# Autodesk Inventor assembly: BodyStructure
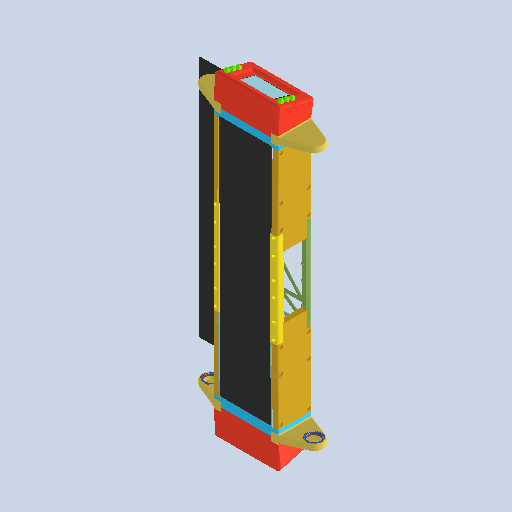
[picture p0: Inventor's stored thumbnail of the model, 512x512]
Saved by Autodesk Inventor 2023 (Build 270158000, 158)
## iProperties
Created: 2022-01-14
Part Number: BodyStructure
Document SubType Name: Assembly
Designer: Jochen
Author: Jochen
## Documents named in this file (13)
- D:\Projects\Lisbeth\CAD\BodyStructure.iam
- D:\Projects\Lisbeth\CAD\Body\BodyStructure Side.ipt
- D:\Projects\Lisbeth\CAD\Body\BodyStructure HipSupport.ipt
- D:\Projects\Lisbeth\CAD\Body\BodyStructure Centre Top.ipt
- D:\Projects\Lisbeth\CAD\Body\BodyStructure Plate.ipt
- D:\Projects\Lisbeth\CAD\Common\Bearing\bearing_27_20_4 s61704-2rsr.ipt
- D:\Projects\Lisbeth\CAD\Body\BodyCover.ipt
- D:\Projects\Lisbeth\CAD\Common\Accessories\Battery Pack.ipt
- D:\Projects\Lisbeth\CAD\Body\BodyStructure Centre Bottom.ipt
- D:\Projects\Lisbeth\CAD\Body\BodyStructure Head.ipt
- D:\Projects\Lisbeth\CAD\Body\BodyStructure Tail.ipt
- D:\Projects\Lisbeth\CAD\Common\Accessories\Adafruit 2.4 OLED display.ipt
- D:\Projects\Lisbeth\CAD\Common\Accessories\LED 5mm.ipt
## Components (28 placed, 10 different names)
1. BodyStructure Side:1 — Mate:89, Mate:100, Mate:102, Mate:142, Mate:149, Mate:150
2. BodyStructure Side:2 — Mate:109, Mate:110, Mate:111, Mate:138, Mate:139, Mate:140
3. BodyHipSupport:1 — Mate:38, Mate:39, Mate:153, Mate:154
4. BodyHipSupport:2 — Mate:44, Mate:45, Mate:151, Mate:152
5. Body Structure Centre Top:2 — Mate:46, Mate:95, Mate:115, Mate:116, Mate:138, Mate:140
6. BodyStructure Side:3 — Mate:46, Angle:2, Mate:139, Mate:141, Mate:143, Mate:144
7. BodyStructure Side:4 — Mate:101, Mate:115, Mate:142
8. BodyHipSupport:3 — Mate:42, Mate:43, Mate:145, Mate:146
9. BodyHipSupport:4 — Mate:40, Mate:41, Mate:147, Mate:148
10. bearing_27_20_4 s61704-2rsr:1 — Mate:38, Mate:39
11. bearing_27_20_4 s61704-2rsr:2 — Mate:44, Mate:45
12. bearing_27_20_4 s61704-2rsr:3 — Mate:40, Mate:41
13. bearing_27_20_4 s61704-2rsr:4 — Mate:42, Mate:43
14. BodyCover:1 — Mate:103, Mate:113
15. BodyCover:2 — Mate:95, Mate:116, Angle:1
16. Battery Pack 59x31x21:1 — Angle:1, Angle:2, Mate:159
17. Body Structure Centre:7 — Mate:89, Mate:109
18. Body Structure Centre Top:1 — Mate:100, Mate:101, Mate:102, Mate:103, Mate:113, Mate:141
19. Body Structure Centre:9 — Mate:110, Mate:111
20. BodyStructure Head:4 — Mate:143, Mate:144, Mate:145, Mate:146, Mate:147, Mate:148, Flush:1, Mate:156, Mate:157, Mate:158, Mate:159, Mate:160, Mate:161, Mate:162, Mate:163, Mate:164, Mate:165, Mate:166, Mate:167, Mate:168, Mate:169, Mate:170, Mate:171, Mate:172
21. BodyStructure Head:5 — Mate:149, Mate:150, Mate:151, Mate:152, Mate:153, Mate:154
22. Adafruit 2.4 OLED display:1 — Flush:1, Mate:156, Mate:157, Mate:158
23. LED 5mm:1 — Mate:160, Mate:168, Mate:172
24. LED 5mm:2 — Mate:161, Mate:166
25. LED 5mm:3 — Mate:164, Mate:170
26. LED 5mm:6 — Mate:162, Mate:167
27. LED 5mm:7 — Mate:163, Mate:171
28. LED 5mm:8 — Mate:165, Mate:169
## Relationships (58: Mate 55, Angle 2, Flush 1)
- Mate:38: BodyHipSupport:1 ↔ bearing_27_20_4 s61704-2rsr:1
- Mate:39: BodyHipSupport:1 ↔ bearing_27_20_4 s61704-2rsr:1
- Mate:40: BodyHipSupport:4 ↔ bearing_27_20_4 s61704-2rsr:3
- Mate:41: BodyHipSupport:4 ↔ bearing_27_20_4 s61704-2rsr:3
- Mate:42: BodyHipSupport:3 ↔ bearing_27_20_4 s61704-2rsr:4
- Mate:43: BodyHipSupport:3 ↔ bearing_27_20_4 s61704-2rsr:4
- Mate:44: BodyHipSupport:2 ↔ bearing_27_20_4 s61704-2rsr:2
- Mate:45: BodyHipSupport:2 ↔ bearing_27_20_4 s61704-2rsr:2
- Mate:46: Body Structure Centre Top:2 ↔ BodyStructure Side:3
- Mate:89: BodyStructure Side:1 ↔ Body Structure Centre:7
- Mate:95: Body Structure Centre Top:2 ↔ BodyCover:2
- Mate:100: BodyStructure Side:1 ↔ Body Structure Centre Top:1
- Mate:101: BodyStructure Side:4 ↔ Body Structure Centre Top:1
- Mate:102: BodyStructure Side:1 ↔ Body Structure Centre Top:1
- Mate:103: BodyCover:1 ↔ Body Structure Centre Top:1
- Mate:109: BodyStructure Side:2 ↔ Body Structure Centre:7
- Mate:110: BodyStructure Side:2 ↔ Body Structure Centre:9
- Mate:111: BodyStructure Side:2 ↔ Body Structure Centre:9
- Mate:113: BodyCover:1 ↔ Body Structure Centre Top:1
- Mate:115: Body Structure Centre Top:2 ↔ BodyStructure Side:4
- Mate:116: Body Structure Centre Top:2 ↔ BodyCover:2
- Angle:1 (0 deg): BodyCover:2 ↔ Battery Pack 59x31x21:1
- Angle:2 (0 deg): BodyStructure Side:3 ↔ Battery Pack 59x31x21:1
- Mate:138: BodyStructure Side:2 ↔ Body Structure Centre Top:2
- Mate:139: BodyStructure Side:2 ↔ BodyStructure Side:3
- Mate:140: BodyStructure Side:2 ↔ Body Structure Centre Top:2
- Mate:141: BodyStructure Side:3 ↔ Body Structure Centre Top:1
- Mate:142: BodyStructure Side:1 ↔ BodyStructure Side:4
- Mate:143: BodyStructure Side:3 ↔ BodyStructure Head:4
- Mate:144: BodyStructure Side:3 ↔ BodyStructure Head:4
- Mate:145: BodyHipSupport:3 ↔ BodyStructure Head:4
- Mate:146: BodyHipSupport:3 ↔ BodyStructure Head:4
- Mate:147: BodyHipSupport:4 ↔ BodyStructure Head:4
- Mate:148: BodyHipSupport:4 ↔ BodyStructure Head:4
- Mate:149: BodyStructure Side:1 ↔ BodyStructure Head:5
- Mate:150: BodyStructure Side:1 ↔ BodyStructure Head:5
- Mate:151: BodyHipSupport:2 ↔ BodyStructure Head:5
- Mate:152: BodyHipSupport:2 ↔ BodyStructure Head:5
- Mate:153: BodyHipSupport:1 ↔ BodyStructure Head:5
- Mate:154: BodyHipSupport:1 ↔ BodyStructure Head:5
- Flush:1: BodyStructure Head:4 ↔ Adafruit 2.4 OLED display:1
- Mate:156: BodyStructure Head:4 ↔ Adafruit 2.4 OLED display:1
- Mate:157 (0.25 mm): BodyStructure Head:4 ↔ Adafruit 2.4 OLED display:1
- Mate:158 (0.125 mm): BodyStructure Head:4 ↔ Adafruit 2.4 OLED display:1
- Mate:159: Battery Pack 59x31x21:1 ↔ BodyStructure Head:4
- Mate:160: BodyStructure Head:4 ↔ LED 5mm:1
- Mate:161: BodyStructure Head:4 ↔ LED 5mm:2
- Mate:162: BodyStructure Head:4 ↔ LED 5mm:6
- Mate:163: BodyStructure Head:4 ↔ LED 5mm:7
- Mate:164: BodyStructure Head:4 ↔ LED 5mm:3
- Mate:165: BodyStructure Head:4 ↔ LED 5mm:8
- Mate:166: BodyStructure Head:4 ↔ LED 5mm:2
- Mate:167: BodyStructure Head:4 ↔ LED 5mm:6
- Mate:168: BodyStructure Head:4 ↔ LED 5mm:1
- Mate:169: BodyStructure Head:4 ↔ LED 5mm:8
- Mate:170: BodyStructure Head:4 ↔ LED 5mm:3
- Mate:171: BodyStructure Head:4 ↔ LED 5mm:7
- Mate:172: BodyStructure Head:4 ↔ LED 5mm:1
